# Autodesk Inventor assembly: Actuator_MGN-BG
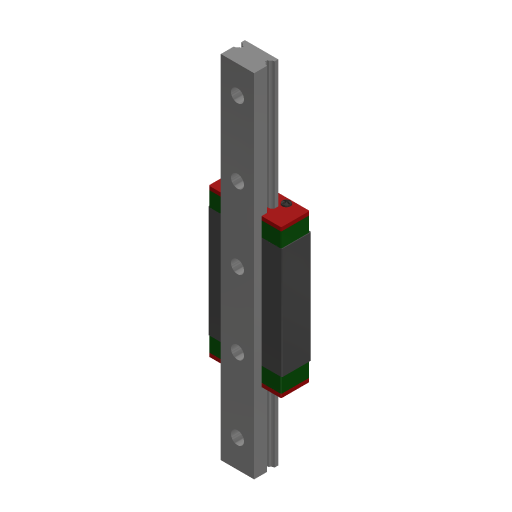
[picture p0: Inventor's stored thumbnail of the model, 512x512]
Saved by Autodesk Inventor 2024.3 (Build 283343000, 343)
## iProperties
Created: 2024-09-13
Part Number: Actuator_MGN-BG
Document SubType Name: Assembly
Designer: Martin
Author: Martin
## Documents named in this file (3)
- D:\User\Dokumente\GitHub\openUC2-OT2-PlateGripper\INVENTOR\Actuator_MGN-BG.iam
- D:\User\Dokumente\GitHub\openUC2-OT2-PlateGripper\INVENTOR\Actuator_MGN9C.ipt
- D:\User\Dokumente\GitHub\openUC2-OT2-PlateGripper\INVENTOR\Actuator_MGN9.ipt
## Components (2 placed, 2 different names)
1. Actuator_MGN9C:1 — Fluchtend:1, Passend:1, Fluchtend:5
2. Actuator_MGN9:1 — Fluchtend:1, Passend:1, Fluchtend:2, Fluchtend:3, Fluchtend:4, Fluchtend:5
## Relationships (6: Flush 5, Mate 1)
- Fluchtend:1 [Flush]: Actuator_MGN9C:1 ↔ Actuator_MGN9:1
- Passend:1 [Mate] (-10 mm): Actuator_MGN9C:1 ↔ Actuator_MGN9:1
- Fluchtend:2 [Flush]: Actuator_MGN9:1
- Fluchtend:3 [Flush]: Actuator_MGN9:1
- Fluchtend:4 [Flush]: Actuator_MGN9:1
- Fluchtend:5 [Flush]: Actuator_MGN9C:1 ↔ Actuator_MGN9:1
